# Autodesk Inventor assembly: drive_left
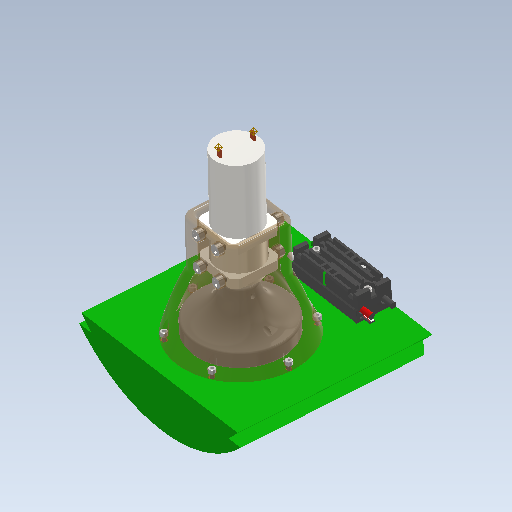
[picture p0: Inventor's stored thumbnail of the model, 512x512]
Saved by Autodesk Inventor 2020.2 (Build 242310000, 310)
## iProperties
Created: 2019-11-08
Part Number: drive_left
Document SubType Name: Assembly
Designer: agmle
Mass: 1199.22 g
Surface Area: 2338.75 cm^2
Volume: 994.04 cm^3
Density: 1.20641 g/cm^3
Author: agmle
## Documents named in this file (17)
- D:\projects\CreekFleet_AutoBuoy\Mechanical CAD\propulsion\drive_left.iam
- D:\projects\CreekFleet_AutoBuoy\Mechanical CAD\propulsion\impeller_left.ipt
- D:\projects\CreekFleet_AutoBuoy\Mechanical CAD\propulsion\drive_disc.ipt
- D:\projects\CreekFleet_AutoBuoy\Mechanical CAD\propulsion\6x10mm magnet.ipt
- D:\projects\CreekFleet_AutoBuoy\Mechanical CAD\propulsion\shaft.ipt
- D:\projects\CreekFleet_AutoBuoy\Mechanical CAD\propulsion\intake_cover.ipt
- D:\projects\CreekFleet_AutoBuoy\Mechanical CAD\propulsion\bearing\6138k63.iam
- \\rackstation\media\documents\Inventor\Content Center Files\R2020\en-US\ANSI B18.3.6M(01)\ANSI B18.3.6M - M3x0.5 x 5(2).ipt
- D:\projects\CreekFleet_AutoBuoy\Mechanical CAD\94459A140_BRASS HEAT-SET INSERT FOR PLASTIC.ipt
- D:\projects\CreekFleet_AutoBuoy\Mechanical CAD\propulsion\rs550_p60s-4-57.ipt
- D:\projects\CreekFleet_AutoBuoy\Mechanical CAD\propulsion\motor_mount.ipt
- \\rackstation\media\documents\Inventor\Content Center Files\R2020\en-US\ANSI B18.3(05)\ANSI B18.3 - 10-32 UNF - 0.5(31).ipt
- D:\projects\CreekFleet_AutoBuoy\Mechanical CAD\propulsion\inner_drive_left.ipt
- \\rackstation\media\documents\Inventor\Content Center Files\R2020\en-US\ANSI B18.3.1M(6)\ANSI B18.3.1M - M3x0.5 x 8(1).ipt
- D:\projects\CreekFleet_AutoBuoy\Mechanical CAD\propulsion\discharge_sealant.ipt
- D:\projects\CreekFleet_AutoBuoy\Mechanical CAD\propulsion\victor spVictor_SP_217-9090_No_Wires.ipt
- \\rackstation\media\documents\Inventor\Content Center Files\R2020\en-US\ANSI B18.3.1M(6)\ANSI B18.3.1M - M3x0.5 x 16(1).ipt
## Components (59 placed, 16 different names)
1. impeller_left:1 — Insert:23, Insert:24, Insert:25, Insert:26, Insert:27, Insert:28, Cylindrical:1, Mate:7, Mate:8
2. 6x10mm magnet:7 — Insert:23
3. 6x10mm magnet:8 — Insert:24
4. 6x10mm magnet:9 — Insert:25
5. 6x10mm magnet:10 — Insert:26
6. 6x10mm magnet:11 — Insert:28
7. 6x10mm magnet:12 — Insert:27
8. shaft:1 — Insert:85, Insert:86, Cylindrical:1
9. 6138k63:1 [sub-assembly] — Insert:84, Insert:85, Mate:7
10. 6138k63:2 [sub-assembly] — Insert:86
11. Broached Hexagon Socket Set Screw - Flat Point - Metric M3x0.5 x 5:1 — Insert:15
12. Broached Hexagon Socket Set Screw - Flat Point - Metric M3x0.5 x 5:2 — Insert:16
13. drive_disc:1 — Insert:15, Insert:16, Insert:17, Insert:18, Insert:19, Insert:20, Insert:21, Insert:22, Mate:1, Mate:3, Mate:8, Flush:1
14. 6x10mm magnet:1 — Insert:21
15. 6x10mm magnet:2 — Insert:20
16. 6x10mm magnet:3 — Insert:19
17. 6x10mm magnet:4 — Insert:18
18. 6x10mm magnet:5 — Insert:17
19. 6x10mm magnet:6 — Insert:22
20. 94459A140_BRASS HEAT-SET INSERT FOR PLASTIC:21 — Insert:105
21. 94459A140_BRASS HEAT-SET INSERT FOR PLASTIC:22 — Insert:104
22. victor spVictor_SP_217-9090_No_Wires:1 — Insert:106, Insert:107, Insert:108, Insert:109
23. Forged Socket Head Cap Screw - Metric M3x0.5 x 16:1 — Insert:108
24. Forged Socket Head Cap Screw - Metric M3x0.5 x 16:2 — Insert:109
25. 94459A140_BRASS HEAT-SET INSERT FOR PLASTIC:15 — Insert:103
26. 94459A140_BRASS HEAT-SET INSERT FOR PLASTIC:16 — Insert:102
27. 94459A140_BRASS HEAT-SET INSERT FOR PLASTIC:17 — Insert:101
28. 94459A140_BRASS HEAT-SET INSERT FOR PLASTIC:18 — Insert:100
29. 94459A140_BRASS HEAT-SET INSERT FOR PLASTIC:19 — Insert:68
30. 94459A140_BRASS HEAT-SET INSERT FOR PLASTIC:20 — Insert:69
31. Forged Socket Head Cap Screw - Metric M3x0.5 x 8:6 — Insert:75
32. Forged Socket Head Cap Screw - Metric M3x0.5 x 8:7 — Insert:74
33. Forged Socket Head Cap Screw - Metric M3x0.5 x 8:8 — Insert:70
34. Forged Socket Head Cap Screw - Metric M3x0.5 x 8:9 — Insert:71
35. Forged Socket Head Cap Screw - Metric M3x0.5 x 8:10 — Insert:73
36. Forged Socket Head Cap Screw - Metric M3x0.5 x 8:11 — Insert:72
37. rs550_p60s-4-57:1 — Mate:1, Mate:2, Mate:3, Flush:1, Mate:9, Mate:10
38. motor_mount:1 — Insert:68, Insert:69, Insert:70, Insert:71, Insert:72, Insert:73, Insert:74, Insert:75, Mate:2, Insert:76, Insert:77, Insert:78, Insert:79, Insert:80, Insert:81, Insert:82, Insert:83, Mate:10, Insert:99
39. Hexagon Socket Head Cap Screw - Inch 10-32 UNF - 0.5:1 — Insert:80
40. Hexagon Socket Head Cap Screw - Inch 10-32 UNF - 0.5:2 — Insert:76
41. Hexagon Socket Head Cap Screw - Inch 10-32 UNF - 0.5:3 — Insert:77
42. Hexagon Socket Head Cap Screw - Inch 10-32 UNF - 0.5:4 — Insert:79
43. Hexagon Socket Head Cap Screw - Inch 10-32 UNF - 0.5:5 — Insert:81
44. Hexagon Socket Head Cap Screw - Inch 10-32 UNF - 0.5:6 — Insert:82, Mate:9
45. Hexagon Socket Head Cap Screw - Inch 10-32 UNF - 0.5:7 — Insert:83
46. Hexagon Socket Head Cap Screw - Inch 10-32 UNF - 0.5:8 — Insert:78
47. discharge_sealant:1 — Mate:11, Mate:12
48. 94459A140_BRASS HEAT-SET INSERT FOR PLASTIC:1 — Insert:91
49. 94459A140_BRASS HEAT-SET INSERT FOR PLASTIC:3 — Insert:88
50. 94459A140_BRASS HEAT-SET INSERT FOR PLASTIC:4 — Insert:90
51. 94459A140_BRASS HEAT-SET INSERT FOR PLASTIC:5 — Insert:89
52. 94459A140_BRASS HEAT-SET INSERT FOR PLASTIC:6 — Insert:87
53. intake_cover:1 — Insert:92, Insert:93, Insert:94, Insert:95, Insert:96, Insert:97, Insert:98
54. Forged Socket Head Cap Screw - Metric M3x0.5 x 8:1 — Insert:95
55. Forged Socket Head Cap Screw - Metric M3x0.5 x 8:2 — Insert:98
56. Forged Socket Head Cap Screw - Metric M3x0.5 x 8:3 — Insert:94
57. Forged Socket Head Cap Screw - Metric M3x0.5 x 8:4 — Insert:97
58. Forged Socket Head Cap Screw - Metric M3x0.5 x 8:5 — Insert:96
59. inner_drive_left:1 — Mate:4, Mate:5, Mate:6, Insert:84, Insert:87, Insert:88, Insert:89, Insert:90, Insert:91, Insert:92, Insert:93, Insert:99, Insert:100, Insert:101, Insert:102, Insert:103, Mate:11, Mate:12, Insert:104, Insert:105, Insert:106, Insert:107
## Relationships (70: Insert 56, Mate 12, CylindricalJoint 1, Flush 1)
- Insert:15: Broached Hexagon Socket Set Screw - Flat Point - Metric M3x0.5 x 5:1 ↔ drive_disc:1
- Insert:16: Broached Hexagon Socket Set Screw - Flat Point - Metric M3x0.5 x 5:2 ↔ drive_disc:1
- Insert:17: drive_disc:1 ↔ 6x10mm magnet:5
- Insert:18: drive_disc:1 ↔ 6x10mm magnet:4
- Insert:19: drive_disc:1 ↔ 6x10mm magnet:3
- Insert:20: drive_disc:1 ↔ 6x10mm magnet:2
- Insert:21: drive_disc:1 ↔ 6x10mm magnet:1
- Insert:22: drive_disc:1 ↔ 6x10mm magnet:6
- Insert:23: impeller_left:1 ↔ 6x10mm magnet:7
- Insert:24: impeller_left:1 ↔ 6x10mm magnet:8
- Insert:25: impeller_left:1 ↔ 6x10mm magnet:9
- Insert:26: impeller_left:1 ↔ 6x10mm magnet:10
- Insert:27: impeller_left:1 ↔ 6x10mm magnet:12
- Insert:28: impeller_left:1 ↔ 6x10mm magnet:11
- Mate:1: drive_disc:1 ↔ rs550_p60s-4-57:1
- Insert:68: 94459A140_BRASS HEAT-SET INSERT FOR PLASTIC:19 ↔ motor_mount:1
- Insert:69: 94459A140_BRASS HEAT-SET INSERT FOR PLASTIC:20 ↔ motor_mount:1
- Insert:70: Forged Socket Head Cap Screw - Metric M3x0.5 x 8:8 ↔ motor_mount:1
- Insert:71: Forged Socket Head Cap Screw - Metric M3x0.5 x 8:9 ↔ motor_mount:1
- Insert:72: Forged Socket Head Cap Screw - Metric M3x0.5 x 8:11 ↔ motor_mount:1
- Insert:73: Forged Socket Head Cap Screw - Metric M3x0.5 x 8:10 ↔ motor_mount:1
- Insert:74: Forged Socket Head Cap Screw - Metric M3x0.5 x 8:7 ↔ motor_mount:1
- Insert:75: Forged Socket Head Cap Screw - Metric M3x0.5 x 8:6 ↔ motor_mount:1
- Mate:2: rs550_p60s-4-57:1 ↔ motor_mount:1
- Mate:3: drive_disc:1 ↔ rs550_p60s-4-57:1
- Insert:76: motor_mount:1 ↔ Hexagon Socket Head Cap Screw - Inch 10-32 UNF - 0.5:2
- Insert:77: motor_mount:1 ↔ Hexagon Socket Head Cap Screw - Inch 10-32 UNF - 0.5:3
- Insert:78: motor_mount:1 ↔ Hexagon Socket Head Cap Screw - Inch 10-32 UNF - 0.5:8
- Insert:79: motor_mount:1 ↔ Hexagon Socket Head Cap Screw - Inch 10-32 UNF - 0.5:4
- Insert:80: motor_mount:1 ↔ Hexagon Socket Head Cap Screw - Inch 10-32 UNF - 0.5:1
- Insert:81: motor_mount:1 ↔ Hexagon Socket Head Cap Screw - Inch 10-32 UNF - 0.5:5
- Insert:82: motor_mount:1 ↔ Hexagon Socket Head Cap Screw - Inch 10-32 UNF - 0.5:6
- Insert:83: motor_mount:1 ↔ Hexagon Socket Head Cap Screw - Inch 10-32 UNF - 0.5:7
- Mate:4: inner_drive_left:1
- Mate:5: inner_drive_left:1
- Mate:6: inner_drive_left:1
- Insert:84: 6138k63:1 ↔ inner_drive_left:1
- Insert:85: shaft:1 ↔ 6138k63:1
- Insert:86: shaft:1 ↔ 6138k63:2
- Cylindrical:1: impeller_left:1 ↔ shaft:1
- Mate:7: impeller_left:1 ↔ 6138k63:1
- Mate:8: impeller_left:1 ↔ drive_disc:1
- Insert:87: 94459A140_BRASS HEAT-SET INSERT FOR PLASTIC:6 ↔ inner_drive_left:1
- Insert:88: 94459A140_BRASS HEAT-SET INSERT FOR PLASTIC:3 ↔ inner_drive_left:1
- Insert:89: 94459A140_BRASS HEAT-SET INSERT FOR PLASTIC:5 ↔ inner_drive_left:1
- Insert:90: 94459A140_BRASS HEAT-SET INSERT FOR PLASTIC:4 ↔ inner_drive_left:1
- Insert:91: 94459A140_BRASS HEAT-SET INSERT FOR PLASTIC:1 ↔ inner_drive_left:1
- Insert:92: intake_cover:1 ↔ inner_drive_left:1
- Insert:93: intake_cover:1 ↔ inner_drive_left:1
- Insert:94: intake_cover:1 ↔ Forged Socket Head Cap Screw - Metric M3x0.5 x 8:3
- Insert:95: intake_cover:1 ↔ Forged Socket Head Cap Screw - Metric M3x0.5 x 8:1
- Insert:96: intake_cover:1 ↔ Forged Socket Head Cap Screw - Metric M3x0.5 x 8:5
- Insert:97: intake_cover:1 ↔ Forged Socket Head Cap Screw - Metric M3x0.5 x 8:4
- Insert:98: intake_cover:1 ↔ Forged Socket Head Cap Screw - Metric M3x0.5 x 8:2
- Flush:1: drive_disc:1 ↔ rs550_p60s-4-57:1
- Mate:9: rs550_p60s-4-57:1 ↔ Hexagon Socket Head Cap Screw - Inch 10-32 UNF - 0.5:6
- Mate:10: rs550_p60s-4-57:1 ↔ motor_mount:1
- Insert:99: motor_mount:1 ↔ inner_drive_left:1
- Insert:100: 94459A140_BRASS HEAT-SET INSERT FOR PLASTIC:18 ↔ inner_drive_left:1
- Insert:101: 94459A140_BRASS HEAT-SET INSERT FOR PLASTIC:17 ↔ inner_drive_left:1
- Insert:102: 94459A140_BRASS HEAT-SET INSERT FOR PLASTIC:16 ↔ inner_drive_left:1
- Insert:103: 94459A140_BRASS HEAT-SET INSERT FOR PLASTIC:15 ↔ inner_drive_left:1
- Mate:11: discharge_sealant:1 ↔ inner_drive_left:1
- Mate:12: discharge_sealant:1 ↔ inner_drive_left:1
- Insert:104: 94459A140_BRASS HEAT-SET INSERT FOR PLASTIC:22 ↔ inner_drive_left:1
- Insert:105: 94459A140_BRASS HEAT-SET INSERT FOR PLASTIC:21 ↔ inner_drive_left:1
- Insert:106: victor spVictor_SP_217-9090_No_Wires:1 ↔ inner_drive_left:1
- Insert:107: victor spVictor_SP_217-9090_No_Wires:1 ↔ inner_drive_left:1
- Insert:108: victor spVictor_SP_217-9090_No_Wires:1 ↔ Forged Socket Head Cap Screw - Metric M3x0.5 x 16:1
- Insert:109: victor spVictor_SP_217-9090_No_Wires:1 ↔ Forged Socket Head Cap Screw - Metric M3x0.5 x 16:2
